# Autodesk Inventor assembly: Assembly
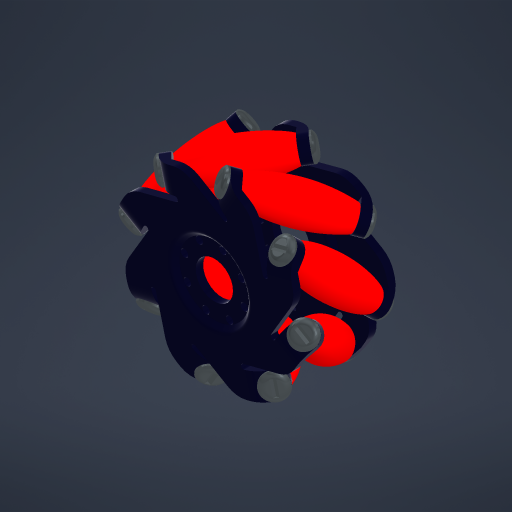
[picture p0: Inventor's stored thumbnail of the model, 512x512]
Saved by Autodesk Inventor 2023 (Build 270158000, 158)
## iProperties
Created: 2023-04-05
Part Number: Assembly
Document SubType Name: Assembly
Designer: vatdu
Author: vatdu
## Documents named in this file (4)
- C:\Users\vatdu\Desktop\CRYSTAL MARK II\Wheels\Mecanum Wheel.iam
- C:\Users\vatdu\Desktop\CRYSTAL MARK II\Wheels\Roller V3.ipt
- C:\Users\vatdu\Desktop\CRYSTAL MARK II\Wheels\Frame V2.ipt
- C:\Users\vatdu\Desktop\CRYSTAL MARK II\Components\Screw.ipt
## Components (26 placed, 3 different names)
1. Roller V3:1 — Rotational:4
2. Roller V3:2 — Rotational:5
3. Roller V3:3 — Rotational:6
4. Roller V3:4 — Rotational:7
5. Roller V3:5 — Rotational:8
6. Roller V3:6 — Rotational:3
7. Roller V3:7 — Rotational:2
8. Roller V3:8 — Rotational:1
9. Frame V2:1 — Rotational:1, Rotational:2, Rotational:3, Rotational:4, Rotational:5, Rotational:6, Rotational:7, Rotational:8, Rotational:9, Rotational:10, Rotational:11, Rotational:12, Rotational:13, Rotational:14, Rotational:15, Rotational:16
10. Frame V2:2 — Rotational:17, Rotational:18, Rotational:19, Rotational:20, Rotational:21, Rotational:22, Rotational:23, Rotational:24
11. Screw:1 — Rotational:9
12. Screw:2 — Rotational:10
13. Screw:3 — Rotational:11
14. Screw:4 — Rotational:12
15. Screw:5 — Rotational:13
16. Screw:6 — Rotational:14
17. Screw:7 — Rotational:16
18. Screw:8 — Rotational:15
19. Screw:9 — Rotational:20
20. Screw:10 — Rotational:22
21. Screw:11 — Rotational:18
22. Screw:12 — Rotational:17
23. Screw:13 — Rotational:21
24. Screw:14 — Rotational:19
25. Screw:15 — Rotational:23
26. Screw:16 — Rotational:24
## Relationships (24: RevoluteJoint 24)
- Rotational:1 [RevoluteJoint]: Roller V3:8 ↔ Frame V2:1
- Rotational:2 [RevoluteJoint]: Roller V3:7 ↔ Frame V2:1
- Rotational:3 [RevoluteJoint]: Roller V3:6 ↔ Frame V2:1
- Rotational:4 [RevoluteJoint]: Roller V3:1 ↔ Frame V2:1
- Rotational:5 [RevoluteJoint]: Roller V3:2 ↔ Frame V2:1
- Rotational:6 [RevoluteJoint]: Roller V3:3 ↔ Frame V2:1
- Rotational:7 [RevoluteJoint]: Roller V3:4 ↔ Frame V2:1
- Rotational:8 [RevoluteJoint]: Roller V3:5 ↔ Frame V2:1
- Rotational:9 [RevoluteJoint]: Frame V2:1 ↔ Screw:1
- Rotational:10 [RevoluteJoint]: Frame V2:1 ↔ Screw:2
- Rotational:11 [RevoluteJoint]: Frame V2:1 ↔ Screw:3
- Rotational:12 [RevoluteJoint]: Frame V2:1 ↔ Screw:4
- Rotational:13 [RevoluteJoint]: Frame V2:1 ↔ Screw:5
- Rotational:14 [RevoluteJoint]: Frame V2:1 ↔ Screw:6
- Rotational:15 [RevoluteJoint]: Frame V2:1 ↔ Screw:8
- Rotational:16 [RevoluteJoint]: Frame V2:1 ↔ Screw:7
- Rotational:17 [RevoluteJoint]: Frame V2:2 ↔ Screw:12
- Rotational:18 [RevoluteJoint]: Frame V2:2 ↔ Screw:11
- Rotational:19 [RevoluteJoint]: Frame V2:2 ↔ Screw:14
- Rotational:20 [RevoluteJoint]: Frame V2:2 ↔ Screw:9
- Rotational:21 [RevoluteJoint]: Frame V2:2 ↔ Screw:13
- Rotational:22 [RevoluteJoint]: Frame V2:2 ↔ Screw:10
- Rotational:23 [RevoluteJoint]: Frame V2:2 ↔ Screw:15
- Rotational:24 [RevoluteJoint]: Frame V2:2 ↔ Screw:16
